# Autodesk Inventor assembly: hodoscopeHolder
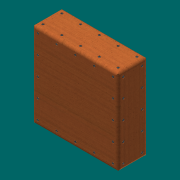
[picture p0: Inventor's stored thumbnail of the model, 180x180]
Saved by Autodesk Inventor 2016 SP1 (Build 200210100, 210)
## iProperties
Created: 2016-02-10
Part Number: hodoscopeHolder
Document SubType Name: Assembly
Designer: Sawaiz
Author: Sawaiz
## Documents named in this file (5)
- C:\Users\sawai\OneDrive\projects\modularHodoscope\hodoscope.iam
- C:\Users\sawai\OneDrive\projects\modularHodoscope\hodoscopeBare.iam
- C:\Users\sawai\OneDrive\projects\modularHodoscope\facing\sideFacing.iam
- C:\Users\sawai\OneDrive\projects\modularHodoscope\facing\frontBackFacing.iam
- C:\Users\sawai\OneDrive\projects\modularHodoscope\facing\matingORing.ipt
## Components (9 placed, 4 different names)
1. hodoscopeBare:1 [sub-assembly] — Mate:1, Flush:1, Flush:2, Mate:2, Flush:3, Mate:5, Flush:4, Flush:5, Mate:6, Mate:16
2. sideFacing:1 [sub-assembly] — Mate:1, Flush:1, Flush:2, Mate:3, Mate:14, Mate:17, Mate:19, Mate:21, Mate:22
3. sideFacing:2 [sub-assembly] — Mate:2, Flush:3, Mate:3, Mate:4, Mate:15
4. sideFacing:3 [sub-assembly] — Mate:4, Mate:5, Flush:4, Mate:7
5. sideFacing:4 [sub-assembly] — Flush:5, Mate:6, Mate:7, Mate:18, Mate:20, Mate:23
6. frontBackFacing:2 [sub-assembly] — Mate:21, Mate:22, Mate:23
7. frontBackFacing:3 [sub-assembly] — Mate:16, Mate:17, Mate:18
8. matingORing:1 — Mate:14, Mate:15
9. matingORing:2 — Mate:19, Mate:20
## Relationships (22: Mate 17, Flush 5)
- Mate:1: hodoscopeBare:1 ↔ sideFacing:1
- Flush:1: hodoscopeBare:1 ↔ sideFacing:1
- Flush:2: hodoscopeBare:1 ↔ sideFacing:1
- Mate:2: hodoscopeBare:1 ↔ sideFacing:2
- Flush:3: hodoscopeBare:1 ↔ sideFacing:2
- Mate:3: sideFacing:1 ↔ sideFacing:2
- Mate:4: sideFacing:2 ↔ sideFacing:3
- Mate:5: hodoscopeBare:1 ↔ sideFacing:3
- Flush:4: hodoscopeBare:1 ↔ sideFacing:3
- Flush:5: hodoscopeBare:1 ↔ sideFacing:4
- Mate:6: hodoscopeBare:1 ↔ sideFacing:4
- Mate:7: sideFacing:3 ↔ sideFacing:4
- Mate:14: sideFacing:1 ↔ matingORing:1
- Mate:15: sideFacing:2 ↔ matingORing:1
- Mate:16: hodoscopeBare:1 ↔ frontBackFacing:3
- Mate:17: sideFacing:1 ↔ frontBackFacing:3
- Mate:18: sideFacing:4 ↔ frontBackFacing:3
- Mate:19: sideFacing:1 ↔ matingORing:2
- Mate:20: sideFacing:4 ↔ matingORing:2
- Mate:21: sideFacing:1 ↔ frontBackFacing:2
- Mate:22: sideFacing:1 ↔ frontBackFacing:2
- Mate:23: sideFacing:4 ↔ frontBackFacing:2
